# Autodesk Inventor assembly: Assembly6
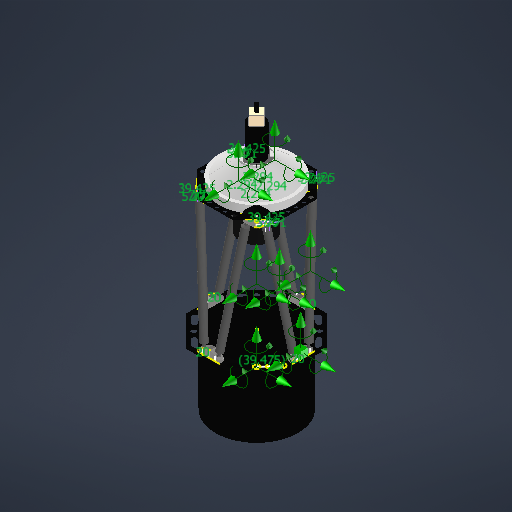
[picture p0: Inventor's stored thumbnail of the model, 512x512]
Saved by Autodesk Inventor 2026.2 (Build 302298000, 298)
## iProperties
Created: 2025-12-09
Part Number: Assembly6
Document SubType Name: Assembly
Designer: Thoma
Author: Thoma
## Documents named in this file (25)
- C:\Users\Thoma\OneDrive\Desktop\Inventor\Quarter_Open\Version_2\Main.iam
- C:\Users\Thoma\OneDrive\Desktop\Inventor\Quarter_Open\Version_2\Telescope_End.ipt
- C:\Users\Thoma\OneDrive\Desktop\Inventor\Quarter_Open\Version_2\Triangle.ipt
- C:\Users\Thoma\OneDrive\Desktop\Inventor\Quarter_Open\Version_2\Triangle_Bracket_Top.ipt
- C:\Users\Thoma\OneDrive\Desktop\Inventor\Quarter_Open\Version_2\Carbon_Fibre.ipt
- C:\Users\Thoma\OneDrive\Desktop\Inventor\Quarter_Open\Version_2\5mm Screw.ipt
- C:\Users\Thoma\OneDrive\Desktop\Inventor\Quarter_Open\Version_2\Triangle_Bracket_Top_MIR.ipt
- C:\Users\Thoma\OneDrive\Desktop\Inventor\Quarter_Open\Version_2\Triangle_MIR.ipt
- C:\Users\Thoma\OneDrive\Desktop\Inventor\Quarter_Open\Version_2\5mm Screw_MIR.ipt
- C:\Users\Thoma\OneDrive\Desktop\Inventor\Quarter_Open\Version_2\Triangle_Bracket_Top_MIR1.ipt
- C:\Users\Thoma\OneDrive\Desktop\Inventor\Quarter_Open\Version_2\Triangle_MIR1.ipt
- C:\Users\Thoma\OneDrive\Desktop\Inventor\Quarter_Open\Version_2\5mm Screw_MIR1.ipt
- C:\Users\Thoma\OneDrive\Desktop\Inventor\Quarter_Open\Version_2\Triangle_Bracket_Top_MIR_MIR.ipt
- C:\Users\Thoma\OneDrive\Desktop\Inventor\Quarter_Open\Version_2\Triangle_MIR_MIR.ipt
- C:\Users\Thoma\OneDrive\Desktop\Inventor\Quarter_Open\Version_2\5mm Screw_MIR_MIR.ipt
- C:\Users\Thoma\OneDrive\Desktop\Inventor\Quarter_Open\Version_2\35mm_bolt.ipt
- C:\Users\Thoma\OneDrive\Desktop\Inventor\Quarter_Open\Version_2\Triangle_Bracket_Bottom_MIR.ipt
- C:\Users\Thoma\OneDrive\Desktop\Inventor\Quarter_Open\Version_2\Telescope_Base.ipt
- C:\Users\Thoma\OneDrive\Desktop\Inventor\Quarter_Open\Version_2\Bottom_End_Top.ipt
- C:\Users\Thoma\OneDrive\Desktop\Inventor\Quarter_Open\Version_2\Full_shaft_Simplify_3.ipt
- C:\Users\Thoma\OneDrive\Desktop\Inventor\Quarter_Open\Version_2\Conic_Cover_Simplify_1.ipt
- C:\Users\Thoma\OneDrive\Desktop\Inventor\Quarter_Open\Version_2\30mm_bolt.ipt
- C:\Users\Thoma\OneDrive\Desktop\Inventor\Quarter_Open\Version_2\Cover_Lower_v3.ipt
- C:\Users\Thoma\OneDrive\Desktop\Inventor\Quarter_Open\Version_2\Cover_Upper_v2.ipt
- C:\Users\Thoma\OneDrive\Desktop\Inventor\Quarter_Open\Version_2\Baffle.ipt
## Components (56 placed, 24 different names)
1. Telescope_End:1 — Mate:1, Mate:2, Angle:2, Mate:7, Mate:20, Mate:21, Angle:11, Mate:30, Mate:31, Angle:18, Mate:40, Mate:41, Angle:21, Mate:54, Mate:55, Mate:56, Mate:57, Angle:26, Angle:31, Angle:41
2. Triangle_Bracket_Top:1 — Mate:1, Mate:2, Angle:2, Mate:8, Mate:9, Angle:4, Mate:47, Angle:22, Mate:58, Tangent:7
3. Carbon_Fibre:1 — Mate:7, Mate:11, Flush:1, Mate:12, Mate:13, Mate:14, Mate:15, Mate:22, Mate:23, Mate:24, Mate:25, Mate:32, Mate:33, Mate:34, Mate:35, Mate:42, Mate:43, Mate:44, Mate:45, Mate:62, Flush:2, Flush:3, Flush:4, Flush:5, Mate:83
4. Triangle:1 — Mate:8, Mate:9, Angle:4, Mate:11, Flush:1, Angle:5, Angle:6, Mate:46, Mate:70, Mate:71
5. 5mm Screw:1 — Mate:12, Mate:13, Angle:5
6. 5mm Screw:2 — Mate:14, Mate:15, Angle:6
7. Triangle_Bracket_Top_MIR:1 — Angle:7, Mate:16, Mate:17, Mate:20, Mate:21, Angle:11, Mate:49, Angle:23, Mate:61, Angle:29, Tangent:5
8. Triangle_MIR:1 — Angle:7, Mate:16, Mate:17, Angle:8, Angle:9, Mate:48, Mate:65, Mate:72, Flush:14
9. 5mm Screw_MIR:1 — Angle:8, Mate:22, Mate:23
10. 5mm Screw_MIR:2 — Angle:9, Mate:24, Mate:25
11. Triangle_Bracket_Top_MIR1:1 — Angle:12, Mate:26, Mate:27, Mate:40, Mate:41, Angle:21, Angle:25, Mate:59, Angle:27, Tangent:6
12. Triangle_MIR1:1 — Angle:12, Mate:26, Mate:27, Angle:13, Angle:14, Mate:52, Mate:53, Mate:68, Mate:69, Flush:83
13. 5mm Screw_MIR1:1 — Angle:13, Mate:42, Mate:43
14. 5mm Screw_MIR1:2 — Angle:14, Mate:44, Mate:45
15. Triangle_Bracket_Top_MIR_MIR:1 — Mate:28, Mate:29, Angle:15, Mate:30, Mate:31, Angle:18, Angle:24, Angle:28, Mate:60, Tangent:8
16. Triangle_MIR_MIR:1 — Mate:28, Mate:29, Angle:15, Angle:16, Angle:17, Mate:50, Mate:51, Mate:66, Mate:67
17. 5mm Screw_MIR_MIR:1 — Angle:16, Mate:32, Mate:33
18. 5mm Screw_MIR_MIR:2 — Angle:17, Mate:34, Mate:35
19. 35mm_bolt:1 — Mate:52, Mate:53, Angle:25
20. 35mm_bolt:2 — Mate:50, Mate:51, Angle:24
21. 35mm_bolt:3 — Mate:48, Mate:49, Angle:23
22. 35mm_bolt:4 — Mate:46, Mate:47, Angle:22
23. Triangle_Bracket_Bottom_MIR:1 — Mate:54, Mate:61, Angle:29, Mate:79, Flush:12, Angle:38, Mate:80, Flush:13, Angle:39, Angle:40, Tangent:9
24. Triangle_Bracket_Bottom_MIR:2 — Mate:55, Mate:58, Angle:26, Tangent:4, Mate:77, Flush:10, Angle:36, Mate:78, Flush:11, Angle:37
25. Triangle_Bracket_Bottom_MIR:3 — Mate:56, Angle:28, Mate:60, Mate:73, Flush:6, Angle:32, Mate:74, Flush:7, Angle:33
26. Triangle_Bracket_Bottom_MIR:4 — Mate:57, Mate:59, Angle:27, Mate:75, Flush:8, Angle:34, Mate:76, Flush:9, Angle:35
27. Telescope_Base:1 — Mate:62, Mate:63, Mate:64, Angle:30, Angle:31, Mate:85
28. Conic_Cover_Simplify_1:1 — Mate:65, Flush:2, Mate:66
29. Conic_Cover_Simplify_1:2 — Mate:67, Flush:3, Mate:68
30. Conic_Cover_Simplify_1:3 — Mate:69, Flush:4, Mate:70
31. Conic_Cover_Simplify_1:4 — Mate:71, Flush:5, Mate:72
32. 30mm_bolt:1 — Mate:73, Flush:6, Angle:32
33. 30mm_bolt:2 — Mate:77, Flush:10, Angle:36
34. 30mm_bolt:3 — Mate:79, Flush:12, Angle:38
35. 30mm_bolt:4 — Mate:75, Flush:8, Angle:34
36. 30mm_bolt:5 — Mate:76, Flush:9, Angle:35
37. 30mm_bolt:6 — Mate:78, Flush:11, Angle:37
38. 30mm_bolt:7 — Mate:74, Flush:7, Angle:33
39. 30mm_bolt:8 — Mate:80, Flush:13, Angle:39
40. Cover_Lower_v3:1 — Flush:14, Tangent:5, Angle:40, Mate:81
41. Cover_Lower_v3:3 — Flush:83, Tangent:6, Angle:41, Mate:82
42. Cover_Upper_v2:1 — Tangent:7, Mate:81
43. Cover_Upper_v2:2 — Tangent:8, Mate:82
44. Baffle:1 — Mate:83, Mate:85
45. Full_shaft_Simplify_3:1 — Tangent:3, Tangent:4
46. Full_shaft_Simplify_3:2 — Tangent:9
47. Bottom_End_Top:1 — Mate:63, Mate:64, Angle:30, Tangent:3
48. Full_shaft_Simplify_3:3
49. Full_shaft_Simplify_3:4
50. Bottom_End_Top:2
51. Full_shaft_Simplify_3:5
52. Full_shaft_Simplify_3:6
53. Bottom_End_Top:3
54. Full_shaft_Simplify_3:7
55. Full_shaft_Simplify_3:8
56. Bottom_End_Top:4
## Component patterns: (4 elements, first: Full_shaft_Simplify_3:1 + Full_shaft_Simplify_3:2 + Bottom_End_Top:1)
## Relationships (131: Mate 73, Angle 36, Flush 15, Tangent 7)
- Mate:1: Telescope_End:1 ↔ Triangle_Bracket_Top:1
- Mate:2: Telescope_End:1 ↔ Triangle_Bracket_Top:1
- Angle:2 (0 deg): Telescope_End:1 ↔ Triangle_Bracket_Top:1
- Mate:7: Telescope_End:1 ↔ Carbon_Fibre:1
- Mate:8: Triangle_Bracket_Top:1 ↔ Triangle:1
- Mate:9: Triangle_Bracket_Top:1 ↔ Triangle:1
- Angle:4 (0 deg): Triangle_Bracket_Top:1 ↔ Triangle:1
- Mate:11: Carbon_Fibre:1 ↔ Triangle:1
- Flush:1: Carbon_Fibre:1 ↔ Triangle:1
- Mate:12: Carbon_Fibre:1 ↔ 5mm Screw:1
- Mate:13: Carbon_Fibre:1 ↔ 5mm Screw:1
- Angle:5 (0 deg): Triangle:1 ↔ 5mm Screw:1
- Mate:14: Carbon_Fibre:1 ↔ 5mm Screw:2
- Mate:15: Carbon_Fibre:1 ↔ 5mm Screw:2
- Angle:6 (0 deg): Triangle:1 ↔ 5mm Screw:2
- Angle:7 (0 deg): Triangle_Bracket_Top_MIR:1 ↔ Triangle_MIR:1
- Mate:16: Triangle_Bracket_Top_MIR:1 ↔ Triangle_MIR:1
- Mate:17: Triangle_Bracket_Top_MIR:1 ↔ Triangle_MIR:1
- Angle:8 (0 deg): Triangle_MIR:1 ↔ 5mm Screw_MIR:1
- Angle:9 (0 deg): Triangle_MIR:1 ↔ 5mm Screw_MIR:2
- Mate:20: Telescope_End:1 ↔ Triangle_Bracket_Top_MIR:1
- Mate:21: Telescope_End:1 ↔ Triangle_Bracket_Top_MIR:1
- Angle:11 (0 deg): Telescope_End:1 ↔ Triangle_Bracket_Top_MIR:1
- Mate:22: Carbon_Fibre:1 ↔ 5mm Screw_MIR:1
- Mate:23: Carbon_Fibre:1 ↔ 5mm Screw_MIR:1
- Mate:24: Carbon_Fibre:1 ↔ 5mm Screw_MIR:2
- Mate:25: Carbon_Fibre:1 ↔ 5mm Screw_MIR:2
- Angle:12 (0 deg): Triangle_Bracket_Top_MIR1:1 ↔ Triangle_MIR1:1
- Mate:26: Triangle_Bracket_Top_MIR1:1 ↔ Triangle_MIR1:1
- Mate:27: Triangle_Bracket_Top_MIR1:1 ↔ Triangle_MIR1:1
- Angle:13 (0 deg): Triangle_MIR1:1 ↔ 5mm Screw_MIR1:1
- Angle:14 (0 deg): Triangle_MIR1:1 ↔ 5mm Screw_MIR1:2
- Mate:28: Triangle_Bracket_Top_MIR_MIR:1 ↔ Triangle_MIR_MIR:1
- Mate:29: Triangle_Bracket_Top_MIR_MIR:1 ↔ Triangle_MIR_MIR:1
- Angle:15 (0 deg): Triangle_Bracket_Top_MIR_MIR:1 ↔ Triangle_MIR_MIR:1
- Angle:16 (0 deg): Triangle_MIR_MIR:1 ↔ 5mm Screw_MIR_MIR:1
- Angle:17 (0 deg): Triangle_MIR_MIR:1 ↔ 5mm Screw_MIR_MIR:2
- Mate:30: Telescope_End:1 ↔ Triangle_Bracket_Top_MIR_MIR:1
- Mate:31: Telescope_End:1 ↔ Triangle_Bracket_Top_MIR_MIR:1
- Angle:18 (0 deg): Telescope_End:1 ↔ Triangle_Bracket_Top_MIR_MIR:1
- Mate:32: Carbon_Fibre:1 ↔ 5mm Screw_MIR_MIR:1
- Mate:33: Carbon_Fibre:1 ↔ 5mm Screw_MIR_MIR:1
- Mate:34: Carbon_Fibre:1 ↔ 5mm Screw_MIR_MIR:2
- Mate:35: Carbon_Fibre:1 ↔ 5mm Screw_MIR_MIR:2
- Mate:40: Telescope_End:1 ↔ Triangle_Bracket_Top_MIR1:1
- Mate:41: Telescope_End:1 ↔ Triangle_Bracket_Top_MIR1:1
- Angle:21 (0 deg): Telescope_End:1 ↔ Triangle_Bracket_Top_MIR1:1
- Mate:42: Carbon_Fibre:1 ↔ 5mm Screw_MIR1:1
- Mate:43: Carbon_Fibre:1 ↔ 5mm Screw_MIR1:1
- Mate:44: Carbon_Fibre:1 ↔ 5mm Screw_MIR1:2
- Mate:45: Carbon_Fibre:1 ↔ 5mm Screw_MIR1:2
- Mate:46: Triangle:1 ↔ 35mm_bolt:4
- Mate:47: Triangle_Bracket_Top:1 ↔ 35mm_bolt:4
- Angle:22 (0 deg): Triangle_Bracket_Top:1 ↔ 35mm_bolt:4
- Mate:48: Triangle_MIR:1 ↔ 35mm_bolt:3
- Mate:49: Triangle_Bracket_Top_MIR:1 ↔ 35mm_bolt:3
- Angle:23 (0 deg): Triangle_Bracket_Top_MIR:1 ↔ 35mm_bolt:3
- Mate:50: Triangle_MIR_MIR:1 ↔ 35mm_bolt:2
- Mate:51: Triangle_MIR_MIR:1 ↔ 35mm_bolt:2
- Angle:24 (0 deg): Triangle_Bracket_Top_MIR_MIR:1 ↔ 35mm_bolt:2
- Mate:52: Triangle_MIR1:1 ↔ 35mm_bolt:1
- Mate:53: Triangle_MIR1:1 ↔ 35mm_bolt:1
- Angle:25 (0 deg): Triangle_Bracket_Top_MIR1:1 ↔ 35mm_bolt:1
- Mate:54: Telescope_End:1 ↔ Triangle_Bracket_Bottom_MIR:1
- Mate:55: Telescope_End:1 ↔ Triangle_Bracket_Bottom_MIR:2
- Mate:56: Telescope_End:1 ↔ Triangle_Bracket_Bottom_MIR:3
- Mate:57: Telescope_End:1 ↔ Triangle_Bracket_Bottom_MIR:4
- Mate:58: Triangle_Bracket_Top:1 ↔ Triangle_Bracket_Bottom_MIR:2
- Angle:26 (0 deg): Telescope_End:1 ↔ Triangle_Bracket_Bottom_MIR:2
- Mate:59: Triangle_Bracket_Top_MIR1:1 ↔ Triangle_Bracket_Bottom_MIR:4
- Angle:27 (0 deg): Triangle_Bracket_Top_MIR1:1 ↔ Triangle_Bracket_Bottom_MIR:4
- Angle:28 (0 deg): Triangle_Bracket_Top_MIR_MIR:1 ↔ Triangle_Bracket_Bottom_MIR:3
- Mate:60: Triangle_Bracket_Top_MIR_MIR:1 ↔ Triangle_Bracket_Bottom_MIR:3
- Mate:61: Triangle_Bracket_Top_MIR:1 ↔ Triangle_Bracket_Bottom_MIR:1
- Angle:29 (0 deg): Triangle_Bracket_Top_MIR:1 ↔ Triangle_Bracket_Bottom_MIR:1
- Mate:62: Carbon_Fibre:1 ↔ Telescope_Base:1
- Mate:63: Telescope_Base:1 ↔ Bottom_End_Top:1
- Mate:64: Telescope_Base:1 ↔ Bottom_End_Top:1
- Angle:30 (0 deg): Telescope_Base:1 ↔ Bottom_End_Top:1
- Angle:31 (0 deg): Telescope_End:1 ↔ Telescope_Base:1
- Tangent:3: Full_shaft_Simplify_3:1 ↔ Bottom_End_Top:1
- Tangent:4: Triangle_Bracket_Bottom_MIR:2 ↔ Full_shaft_Simplify_3:1
- Mate:65: Triangle_MIR:1 ↔ Conic_Cover_Simplify_1:1
- Flush:2: Carbon_Fibre:1 ↔ Conic_Cover_Simplify_1:1
- Mate:66: Triangle_MIR_MIR:1 ↔ Conic_Cover_Simplify_1:1
- Mate:67: Triangle_MIR_MIR:1 ↔ Conic_Cover_Simplify_1:2
- Flush:3: Carbon_Fibre:1 ↔ Conic_Cover_Simplify_1:2
- Mate:68: Triangle_MIR1:1 ↔ Conic_Cover_Simplify_1:2
- Mate:69: Triangle_MIR1:1 ↔ Conic_Cover_Simplify_1:3
- Flush:4: Carbon_Fibre:1 ↔ Conic_Cover_Simplify_1:3
- Mate:70: Triangle:1 ↔ Conic_Cover_Simplify_1:3
- Mate:71: Triangle:1 ↔ Conic_Cover_Simplify_1:4
- Flush:5: Carbon_Fibre:1 ↔ Conic_Cover_Simplify_1:4
- Mate:72: Triangle_MIR:1 ↔ Conic_Cover_Simplify_1:4
- Mate:73: Triangle_Bracket_Bottom_MIR:3 ↔ 30mm_bolt:1
- Flush:6: Triangle_Bracket_Bottom_MIR:3 ↔ 30mm_bolt:1
- Angle:32 (0 deg): Triangle_Bracket_Bottom_MIR:3 ↔ 30mm_bolt:1
- Mate:74: Triangle_Bracket_Bottom_MIR:3 ↔ 30mm_bolt:7
- Flush:7: Triangle_Bracket_Bottom_MIR:3 ↔ 30mm_bolt:7
- Angle:33 (0 deg): Triangle_Bracket_Bottom_MIR:3 ↔ 30mm_bolt:7
- Mate:75: Triangle_Bracket_Bottom_MIR:4 ↔ 30mm_bolt:4
- Flush:8: Triangle_Bracket_Bottom_MIR:4 ↔ 30mm_bolt:4
- Angle:34 (0 deg): Triangle_Bracket_Bottom_MIR:4 ↔ 30mm_bolt:4
- Mate:76: Triangle_Bracket_Bottom_MIR:4 ↔ 30mm_bolt:5
- Flush:9: Triangle_Bracket_Bottom_MIR:4 ↔ 30mm_bolt:5
- Angle:35 (0 deg): Triangle_Bracket_Bottom_MIR:4 ↔ 30mm_bolt:5
- Mate:77: Triangle_Bracket_Bottom_MIR:2 ↔ 30mm_bolt:2
- Flush:10: Triangle_Bracket_Bottom_MIR:2 ↔ 30mm_bolt:2
- Angle:36 (0 deg): Triangle_Bracket_Bottom_MIR:2 ↔ 30mm_bolt:2
- Mate:78: Triangle_Bracket_Bottom_MIR:2 ↔ 30mm_bolt:6
- Flush:11: Triangle_Bracket_Bottom_MIR:2 ↔ 30mm_bolt:6
- Angle:37 (0 deg): Triangle_Bracket_Bottom_MIR:2 ↔ 30mm_bolt:6
- Mate:79: Triangle_Bracket_Bottom_MIR:1 ↔ 30mm_bolt:3
- Flush:12: Triangle_Bracket_Bottom_MIR:1 ↔ 30mm_bolt:3
- Angle:38 (0 deg): Triangle_Bracket_Bottom_MIR:1 ↔ 30mm_bolt:3
- Mate:80: Triangle_Bracket_Bottom_MIR:1 ↔ 30mm_bolt:8
- Flush:13: Triangle_Bracket_Bottom_MIR:1 ↔ 30mm_bolt:8
- Angle:39 (0 deg): Triangle_Bracket_Bottom_MIR:1 ↔ 30mm_bolt:8
- Flush:14: Triangle_MIR:1 ↔ Cover_Lower_v3:1
- Tangent:5 (2 mm): Triangle_Bracket_Top_MIR:1 ↔ Cover_Lower_v3:1
- Angle:40 (0 deg): Triangle_Bracket_Bottom_MIR:1 ↔ Cover_Lower_v3:1
- Flush:83: Triangle_MIR1:1 ↔ Cover_Lower_v3:3
- Tangent:6 (2 mm): Triangle_Bracket_Top_MIR1:1 ↔ Cover_Lower_v3:3
- Angle:41 (0 deg): Telescope_End:1 ↔ Cover_Lower_v3:3
- Tangent:7 (2 mm): Triangle_Bracket_Top:1 ↔ Cover_Upper_v2:1
- Mate:81: Cover_Lower_v3:1 ↔ Cover_Upper_v2:1
- Tangent:8 (2 mm): Triangle_Bracket_Top_MIR_MIR:1 ↔ Cover_Upper_v2:2
- Mate:82: Cover_Lower_v3:3 ↔ Cover_Upper_v2:2
- Mate:83: Carbon_Fibre:1 ↔ Baffle:1
- Mate:85 (20 mm): Telescope_Base:1 ↔ Baffle:1
- Tangent:9: Triangle_Bracket_Bottom_MIR:1 ↔ Full_shaft_Simplify_3:2
